# Autodesk Inventor assembly: Kimpletter ESP Mount Complete
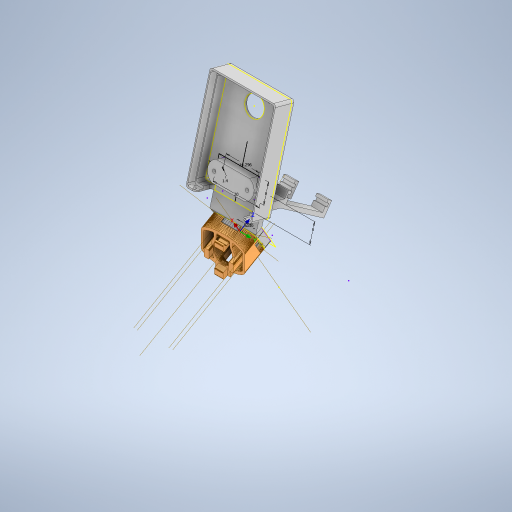
[picture p0: Inventor's stored thumbnail of the model, 512x512]
Saved by Autodesk Inventor 2023 (Build 270158000, 158)
## iProperties
Created: 2023-02-22
Part Number: Kimpletter ESP Mount Complete
Document SubType Name: Assembly
Designer: tommi
Author: tommi
## Documents named in this file (5)
- C:\Users\tommi\Robot_Dog\docs\Inventor\Kimpletter ESP Mount Complete.iam
- C:\Users\tommi\Documents\Inventor\Bittle Upgrades\CAM-Front-Test-V7.ipt
- C:\Users\tommi\Documents\Inventor\Bittle Upgrades\Cam-Neck conection.ipt
- C:\Users\tommi\Documents\Inventor\Bittle Upgrades\Bittle_neck_raw.ipt
- C:\Users\tommi\Documents\Inventor\Bittle Upgrades\ultrasonic-sensor-direct-mount.ipt
## Components (5 placed, 4 different names)
1. CAM-Front-Test-V7:1 — Starr:2
2. Cam-Neck conection:1 — Starr:1, Starr:2, Drehbar:1, Drehbar:2
3. Bittle_neck_raw:1 — Starr:1
4. ultrasonic-sensor-direct-mount:1 — Drehbar:1
5. ultrasonic-sensor-direct-mount:2 — Drehbar:2
## Relationships (4: WeldJoint 2, RevoluteJoint 2)
- Starr:1 [WeldJoint]: Cam-Neck conection:1 ↔ Bittle_neck_raw:1
- Starr:2 [WeldJoint]: CAM-Front-Test-V7:1 ↔ Cam-Neck conection:1
- Drehbar:1 [RevoluteJoint]: Cam-Neck conection:1 ↔ ultrasonic-sensor-direct-mount:1
- Drehbar:2 [RevoluteJoint]: Cam-Neck conection:1 ↔ ultrasonic-sensor-direct-mount:2
